# Autodesk Inventor assembly: ASSY,ROBOT,2026
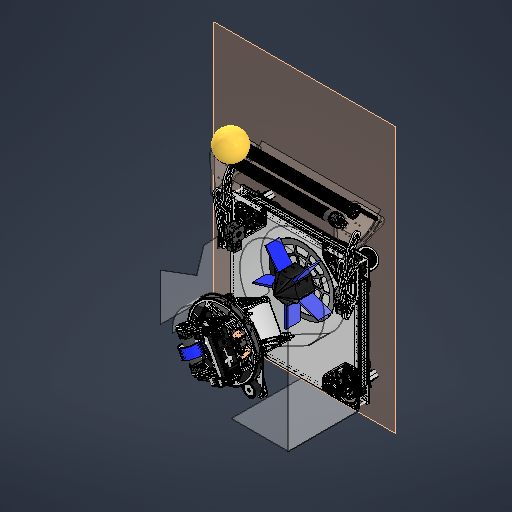
[picture p0: Inventor's stored thumbnail of the model, 512x512]
Saved by Autodesk Inventor 2026 (Build 300175000, 175)
## iProperties
Created: 2026-01-24
Part Number: ASSY,ROBOT,2026
Document SubType Name: Assembly
Designer: Jthib
Mass: 40513.3 g
Surface Area: 94319 cm^2
Volume: 20861.6 cm^3
Density: 1.942 g/cm^3
Author: Jthib
## Documents named in this file (10)
- C:\Users\littl\OneDrive\Documents\GitHub\2026-Robot-Mechanical\ASSY,ROBOT,2026.iam
- C:\Users\littl\OneDrive\Documents\GitHub\2026-Robot-Mechanical\Chassis\CHASSIS.iam
- C:\Users\littl\OneDrive\Documents\GitHub\2026-Robot-Mechanical\Spindexer\#Spindexer.iam
- C:\Users\littl\OneDrive\Documents\GitHub\2026-Robot-Mechanical\Shooter\Shooter - Front Motors\#SHOOTER.FRONT_MOTORS.iam
- C:\Users\littl\OneDrive\Documents\GitHub\2026-Robot-Mechanical\Shooter\Turret\#Turret.iam
- C:\Users\littl\OneDrive\Documents\GitHub\2026-Robot-Mechanical\Intake\ASSY,INTAKE.iam
- C:\Users\littl\OneDrive\Documents\GitHub\2026-Robot-Mechanical\#2_2026 Field CAD\GE-26900_ Fuel.ipt
- C:\Users\littl\OneDrive\Documents\GitHub\2026-Robot-Mechanical\Intake\PLATE,HOPPER,BACK.ipt
- C:\Users\littl\OneDrive\Documents\GitHub\2026-Robot-Mechanical\Intake\PLATE,HOPPER,FRONT.ipt
- C:\Users\littl\OneDrive\Documents\GitHub\2026-Robot-Mechanical\Intake\PLATE,HOPPER,BACK2.ipt
## Components (9 placed, 9 different names)
1. CHASSIS:1 [sub-assembly] — Flush:1, Flush:2, Flush:3, Mate:9, Mate:10, Mate:11, Tangent:1, Mate:13, Mate:18, Mate:19, Mate:20, Mate:21, Flush:23, Mate:22, Flush:24, Mate:23, Mate:25, Flush:25
2. #Spindexer:1 [sub-assembly] — Mate:11, Mate:12, Tangent:1, Mate:13, Mate:15, Mate:16, Mate:17, Mate:18
3. #SHOOTER.FRONT_MOTORS:1 [sub-assembly] — Mate:9, Mate:10, Mate:12, Insert:1, Mate:14
4. #Turret:1 [sub-assembly] — Insert:1, Mate:14, Mate:15, Mate:16, Mate:17
5. ASSY,INTAKE:1 [sub-assembly] — Mate:19, Mate:20, Mate:21
6. GE-26900_ Fuel:1
7. PLATE,HOPPER,BACK:1 — Flush:23, Mate:22, Flush:24, Mate:24
8. PLATE,HOPPER,FRONT:1 — Mate:23, Mate:24
9. PLATE,HOPPER,BACK2:1 — Mate:25, Flush:25
## Relationships (25: Mate 17, Flush 6, Tangent 1, Insert 1)
- Flush:1 (-349.25 mm): CHASSIS:1
- Flush:2 (349.25 mm): CHASSIS:1
- Flush:3: CHASSIS:1
- Mate:9 (-190.5 mm): CHASSIS:1 ↔ #SHOOTER.FRONT_MOTORS:1
- Mate:10 (-190.5 mm): CHASSIS:1 ↔ #SHOOTER.FRONT_MOTORS:1
- Mate:11: CHASSIS:1 ↔ #Spindexer:1
- Mate:12 (79.375 mm): #Spindexer:1 ↔ #SHOOTER.FRONT_MOTORS:1
- Tangent:1: CHASSIS:1 ↔ #Spindexer:1
- Mate:13 (-304.8 mm): CHASSIS:1 ↔ #Spindexer:1
- Insert:1: #SHOOTER.FRONT_MOTORS:1 ↔ #Turret:1
- Mate:14: #SHOOTER.FRONT_MOTORS:1 ↔ #Turret:1
- Mate:15: #Spindexer:1 ↔ #Turret:1
- Mate:16: #Spindexer:1 ↔ #Turret:1
- Mate:17: #Spindexer:1 ↔ #Turret:1
- Mate:18: CHASSIS:1 ↔ #Spindexer:1
- Mate:19: CHASSIS:1 ↔ ASSY,INTAKE:1
- Mate:20: CHASSIS:1 ↔ ASSY,INTAKE:1
- Mate:21: CHASSIS:1 ↔ ASSY,INTAKE:1
- Flush:23: CHASSIS:1 ↔ PLATE,HOPPER,BACK:1
- Mate:22: CHASSIS:1 ↔ PLATE,HOPPER,BACK:1
- Flush:24: CHASSIS:1 ↔ PLATE,HOPPER,BACK:1
- Mate:23: CHASSIS:1 ↔ PLATE,HOPPER,FRONT:1
- Mate:24: PLATE,HOPPER,BACK:1 ↔ PLATE,HOPPER,FRONT:1
- Mate:25: CHASSIS:1 ↔ PLATE,HOPPER,BACK2:1
- Flush:25: CHASSIS:1 ↔ PLATE,HOPPER,BACK2:1
